# Autodesk Inventor assembly: 2AM-17-A-1200 - slider
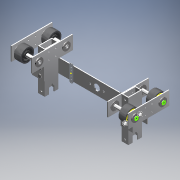
[picture p0: Inventor's stored thumbnail of the model, 180x180]
Saved by Autodesk Inventor 2017 (Build 210142000, 142)
## iProperties
Created: 2017-12-27
Part Number: 2AM-17-A-1200 - slider
Document SubType Name: Assembly
Designer: Micah
Mass: 1647.6 g
Surface Area: 3812.71 cm^2
Volume: 594.036 cm^3
Density: 2.77357 g/cm^3
Author: Micah
## Documents named in this file (10)
- C:\Users\Micah\Desktop\inventor\CADathon-2017\2AM-17-A-0200 - Smokestack Elevator\2AM-17-A-1200 - moving part.iam
- C:\Users\Micah\Desktop\inventor\CADathon-2017\2AM-17-A-0200 - Smokestack Elevator\2AM-17-P-0203 - moving support.ipt
- C:\Users\Micah\Desktop\inventor\CADathon-2017\2AM-17-A-0200 - Smokestack Elevator\2AM-17-P-0205 - moving structure.ipt
- C:\Users\Micah\Desktop\inventor\CADathon-2017\2AM-17-A-0200 - Smokestack Elevator\2AM-17-A-2200 - slider outside.iam
- C:\Users\Micah\Desktop\inventor\CADathon-2017\2AM-17-A-0200 - Smokestack Elevator\2AM-17-A-4200 - inside slider.iam
- C:\Users\Micah\Documents\Inventor\Content Center Files\R2017\en-US\AS 2465(2)\AS 2465 - 1_4 x 1_2  UNC.ipt
- C:\Users\Micah\Documents\Inventor\Content Center Files\R2017\en-US\AS 2465(2)\AS 2465 - 1_4 x 2 1_2  UNC.ipt
- C:\Users\Micah\Documents\Inventor\Content Center Files\R2017\en-US\AS 2465(3)\AS 2465 - 1_4  UNC(2).ipt
- C:\Users\Micah\Desktop\inventor\CADathon-2017\2AM-17-A-0200 - Smokestack Elevator\COTS\217-4399-004 Rev1.ipt
- C:\Users\Micah\Desktop\inventor\CADathon-2017\2AM-17-A-0200 - Smokestack Elevator\2AM-17-P-0206 - moving support slider panl.ipt
## Components (23 placed, 9 different names)
1. 2AM-17-P-0206 - moving support slider panl:1 — Mate:2, Mate:3, Insert:1, Insert:2, Mate:7, Insert:3, Insert:4, Insert:5, Insert:7, Insert:8, Insert:9
2. 2AM-17-P-0203 - moving support:2 — Insert:6, Insert:10, Insert:11, Insert:12, Insert:13, Insert:14, Mate:11, Mate:12, Mate:13, Mate:14, Mate:15, Mate:16, Mate:19
3. 2AM-17-P-0205 - moving structure:2 — Mate:2, Mate:7, Mate:10, Mate:17
4. 2AM-17-P-0205 - moving structure:3 — Mate:3, Mate:9
5. 2AM-17-A-2200 - slider outside:2 [sub-assembly] — Mate:10
6. 2AM-17-A-4200 - inside slider:1 [sub-assembly] — Insert:2, Mate:18, Mate:19
7. 2AM-17-A-4200 - inside slider:2 [sub-assembly] — Insert:1
8. 2AM-17-A-2200 - slider outside:3 [sub-assembly] — Mate:9
9. AS 2465 - Inch 1/4 x 2 1/2  UNC:1 — Insert:3
10. AS 2465 - Inch 1/4 x 2 1/2  UNC:4 — Insert:4
11. AS 2465 - Inch 1/4 x 1/2  UNC:2 — Insert:5
12. AS 2465 - Inch 1/4 x 1/2  UNC:3 — Insert:6
13. AS 2465 - Inch 1/4 x 2 1/2  UNC:3 — Insert:7
14. AS 2465 - Inch 1/4 x 2 1/2  UNC:2 — Insert:8
15. AS 2465 - Inch 1/4 x 1/2  UNC:6 — Insert:9
16. AS 2465 - Inch 1/4 x 1/2  UNC:7 — Insert:10
17. AS 2465 (Unified hexagon bolts, screws and nuts (UNC and UNF threads) - Inch 1/4  UNC:1 — Insert:11
18. AS 2465 (Unified hexagon bolts, screws and nuts (UNC and UNF threads) - Inch 1/4  UNC:2 — Insert:12
19. AS 2465 (Unified hexagon bolts, screws and nuts (UNC and UNF threads) - Inch 1/4  UNC:3 — Insert:13
20. AS 2465 (Unified hexagon bolts, screws and nuts (UNC and UNF threads) - Inch 1/4  UNC:4 — Insert:14
21. 217-4399-004 Rev1:1 — Mate:11, Mate:12, Mate:13
22. 217-4399-004 Rev1:2 — Mate:14, Mate:15, Mate:16
23. 2AM-17-P-0206 - moving support slider panl:3 — Mate:17, Mate:18
## Relationships (28: Mate 14, Insert 14)
- Mate:2: 2AM-17-P-0206 - moving support slider panl:1 ↔ 2AM-17-P-0205 - moving structure:2
- Mate:3: 2AM-17-P-0206 - moving support slider panl:1 ↔ 2AM-17-P-0205 - moving structure:3
- Insert:1: 2AM-17-P-0206 - moving support slider panl:1 ↔ 2AM-17-A-4200 - inside slider:2
- Insert:2: 2AM-17-P-0206 - moving support slider panl:1 ↔ 2AM-17-A-4200 - inside slider:1
- Mate:7: 2AM-17-P-0206 - moving support slider panl:1 ↔ 2AM-17-P-0205 - moving structure:2
- Mate:9: 2AM-17-P-0205 - moving structure:3 ↔ 2AM-17-A-2200 - slider outside:3
- Insert:3: 2AM-17-P-0206 - moving support slider panl:1 ↔ AS 2465 - Inch 1/4 x 2 1/2  UNC:1
- Insert:4: 2AM-17-P-0206 - moving support slider panl:1 ↔ AS 2465 - Inch 1/4 x 2 1/2  UNC:4
- Insert:5: 2AM-17-P-0206 - moving support slider panl:1 ↔ AS 2465 - Inch 1/4 x 1/2  UNC:2
- Insert:6: 2AM-17-P-0203 - moving support:2 ↔ AS 2465 - Inch 1/4 x 1/2  UNC:3
- Insert:7: 2AM-17-P-0206 - moving support slider panl:1 ↔ AS 2465 - Inch 1/4 x 2 1/2  UNC:3
- Insert:8: 2AM-17-P-0206 - moving support slider panl:1 ↔ AS 2465 - Inch 1/4 x 2 1/2  UNC:2
- Insert:9: 2AM-17-P-0206 - moving support slider panl:1 ↔ AS 2465 - Inch 1/4 x 1/2  UNC:6
- Insert:10: 2AM-17-P-0203 - moving support:2 ↔ AS 2465 - Inch 1/4 x 1/2  UNC:7
- Insert:11: 2AM-17-P-0203 - moving support:2 ↔ AS 2465 (Unified hexagon bolts, screws and nuts (UNC and UNF threads) - Inch 1/4  UNC:1
- Insert:12: 2AM-17-P-0203 - moving support:2 ↔ AS 2465 (Unified hexagon bolts, screws and nuts (UNC and UNF threads) - Inch 1/4  UNC:2
- Insert:13: 2AM-17-P-0203 - moving support:2 ↔ AS 2465 (Unified hexagon bolts, screws and nuts (UNC and UNF threads) - Inch 1/4  UNC:3
- Insert:14: 2AM-17-P-0203 - moving support:2 ↔ AS 2465 (Unified hexagon bolts, screws and nuts (UNC and UNF threads) - Inch 1/4  UNC:4
- Mate:10: 2AM-17-P-0205 - moving structure:2 ↔ 2AM-17-A-2200 - slider outside:2
- Mate:11: 2AM-17-P-0203 - moving support:2 ↔ 217-4399-004 Rev1:1
- Mate:12: 2AM-17-P-0203 - moving support:2 ↔ 217-4399-004 Rev1:1
- Mate:13: 2AM-17-P-0203 - moving support:2 ↔ 217-4399-004 Rev1:1
- Mate:14: 2AM-17-P-0203 - moving support:2 ↔ 217-4399-004 Rev1:2
- Mate:15: 2AM-17-P-0203 - moving support:2 ↔ 217-4399-004 Rev1:2
- Mate:16: 2AM-17-P-0203 - moving support:2 ↔ 217-4399-004 Rev1:2
- Mate:17: 2AM-17-P-0205 - moving structure:2 ↔ 2AM-17-P-0206 - moving support slider panl:3
- Mate:18: 2AM-17-A-4200 - inside slider:1 ↔ 2AM-17-P-0206 - moving support slider panl:3
- Mate:19: 2AM-17-P-0203 - moving support:2 ↔ 2AM-17-A-4200 - inside slider:1
